# Autodesk Inventor assembly: 付け根_6_1
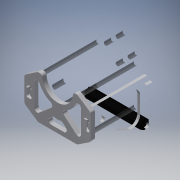
[picture p0: Inventor's stored thumbnail of the model, 180x180]
Saved by Autodesk Inventor 2018 (Build 220112000, 112)
## iProperties
Created: 2016-08-23
Part Number: 付け根_6_1
Material: 一般
Document SubType Name: Assembly
Designer: hiro
Mass: 143.306 g
Surface Area: 289.442 cm^2
Volume: 70.4906 cm^3
Density: 2.03298 g/cm^3
Author: hiro
## Documents named in this file (5)
- Z:\OPR\OpenPlatform_ver1_0\下半身_160823\付け根\付け根_6_1_MIR.iam
- Z:\OPR\OpenPlatform_ver1_0\既製品\B3M11xx.ipt
- Z:\OPR\OpenPlatform_ver1_0\下半身_160823\付け根\付け根_メインフレーム_6_1.ipt
- Z:\OPR\OpenPlatform_ver1_0\下半身_160823\付け根\付け根_サブフレーム_6_1.ipt
- Z:\OPR\OpenPlatform_ver1_0\既製品\新規購入\AMP-340E.ipt
## Components (6 placed, 4 different names)
1. B3M11xx:1 — メイト:1, メイト:2, メイト:3, 挿入:9, 挿入:10, 挿入:11, 挿入:12, 挿入:13, 挿入:14, 挿入:15, 挿入:16
2. 付け根_メインフレーム_6_1:1 — 挿入:13, 挿入:14, 挿入:15, 挿入:16, メイト:8, メイト:9, メイト:10, メイト:11, メイト:12, メイト:13
3. 付け根_サブフレーム_6_1:1 — メイト:7, メイト:10, メイト:11, メイト:13, 挿入:29, 角度:1
4. 付け根_サブフレーム_6_1:2 — メイト:7, メイト:8, メイト:9, メイト:12, 挿入:30
5. 付け根_メインフレーム_6_1:2 — 挿入:9, 挿入:10, 挿入:11, 挿入:12
6. AMP-340E:1 — 挿入:29, 角度:1, 挿入:30
## Relationships (21: Mate 10, Insert 10, Angle 1)
- メイト:1 [Mate] (-19.75 mm): B3M11xx:1
- メイト:2 [Mate] (-25.75 mm): B3M11xx:1
- メイト:3 [Mate] (-16 mm): B3M11xx:1
- メイト:7 [Mate]: 付け根_サブフレーム_6_1:1 ↔ 付け根_サブフレーム_6_1:2
- 挿入:9 [Insert]: B3M11xx:1 ↔ 付け根_メインフレーム_6_1:2
- 挿入:10 [Insert]: B3M11xx:1 ↔ 付け根_メインフレーム_6_1:2
- 挿入:11 [Insert]: B3M11xx:1 ↔ 付け根_メインフレーム_6_1:2
- 挿入:12 [Insert]: B3M11xx:1 ↔ 付け根_メインフレーム_6_1:2
- 挿入:13 [Insert]: B3M11xx:1 ↔ 付け根_メインフレーム_6_1:1
- 挿入:14 [Insert]: B3M11xx:1 ↔ 付け根_メインフレーム_6_1:1
- 挿入:15 [Insert]: B3M11xx:1 ↔ 付け根_メインフレーム_6_1:1
- 挿入:16 [Insert]: B3M11xx:1 ↔ 付け根_メインフレーム_6_1:1
- メイト:8 [Mate] (0.005 mm): 付け根_メインフレーム_6_1:1 ↔ 付け根_サブフレーム_6_1:2
- メイト:9 [Mate] (0.005 mm): 付け根_メインフレーム_6_1:1 ↔ 付け根_サブフレーム_6_1:2
- メイト:10 [Mate] (0.005 mm): 付け根_メインフレーム_6_1:1 ↔ 付け根_サブフレーム_6_1:1
- メイト:11 [Mate] (0.005 mm): 付け根_メインフレーム_6_1:1 ↔ 付け根_サブフレーム_6_1:1
- メイト:12 [Mate]: 付け根_メインフレーム_6_1:1 ↔ 付け根_サブフレーム_6_1:2
- メイト:13 [Mate]: 付け根_メインフレーム_6_1:1 ↔ 付け根_サブフレーム_6_1:1
- 挿入:29 [Insert]: 付け根_サブフレーム_6_1:1 ↔ AMP-340E:1
- 角度:1 [Angle] (0 deg): 付け根_サブフレーム_6_1:1 ↔ AMP-340E:1
- 挿入:30 [Insert]: 付け根_サブフレーム_6_1:2 ↔ AMP-340E:1
## Named parameters: sa_0 = -0, sa_1 = -20000, sa_2 = -1.6e-12
note: some values were not read from the file. Shown as the stored number, unit unknown: "sa_0", "sa_1", "sa_2".
